# Autodesk Inventor assembly: Solenoid
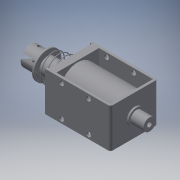
[picture p0: Inventor's stored thumbnail of the model, 180x180]
Saved by Autodesk Inventor 2017 (Build 210142000, 142)
## iProperties
Created: 2017-01-30
Part Number: Solenoid
Document SubType Name: Assembly
Designer: yul067
Author: yul067
## Documents named in this file (5)
- C:\Users\Mike\Desktop\Solenoid 1240S\Solenoid.iam
- C:\Users\Mike\Desktop\Solenoid 1240S\body.ipt
- C:\Users\Mike\Desktop\Solenoid 1240S\cylinder.ipt
- C:\Users\Mike\Desktop\Solenoid 1240S\shaft.ipt
- C:\Users\Mike\Desktop\Solenoid 1240S\spring.ipt
## Components (4 placed, 4 different names)
1. shaft:1 — Cylindrical:1
2. body:1 — Rigid:1, Cylindrical:1, Mate:1
3. cylinder:1 — Rigid:1
4. Spring:1 — Mate:1
## Relationships (3: WeldJoint 1, CylindricalJoint 1, Mate 1)
- Rigid:1 [WeldJoint]: body:1 ↔ cylinder:1
- Cylindrical:1: shaft:1 ↔ body:1
- Mate:1: body:1 ↔ Spring:1
